# Autodesk Inventor assembly: FrontWheelForkAssembly
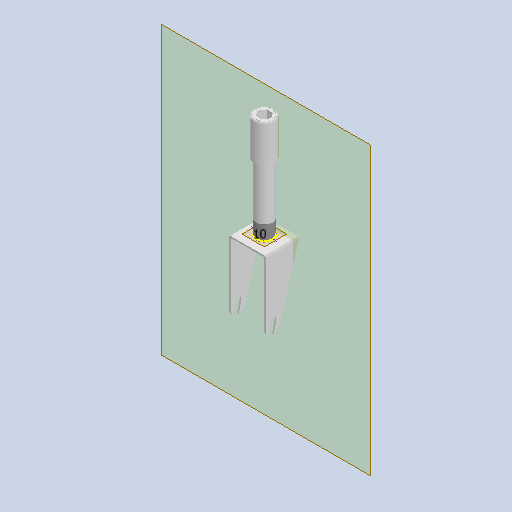
[picture p0: Inventor's stored thumbnail of the model, 512x512]
Saved by Autodesk Inventor 2022.2 (Build 262287000, 287)
## iProperties
Created: 2022-04-13
Part Number: FrontWheelForkAssembly
Document SubType Name: Assembly
Designer: foriw
Mass: 127.99 g
Surface Area: 764.001 cm^2
Volume: 122.116 cm^3
Density: 1.0481 g/cm^3
Author: foriw
## Documents named in this file (6)
- H:\inventor ting\Mekatronik beercart git\Beercart CAD\Workspaces\Workspace\FrontWheelForkAssembly.iam
- H:\inventor ting\Mekatronik beercart git\Beercart CAD\Workspaces\Workspace\Solid2.ipt
- H:\inventor ting\Mekatronik beercart git\Beercart CAD\Workspaces\Workspace\Solid3.ipt
- H:\inventor ting\Mekatronik beercart git\Beercart CAD\Libraries\Content Center Files\en-US\ISO 4762(2)\ISO 4762 - M5 x 12ISO.ipt
- H:\inventor ting\Mekatronik beercart git\Beercart CAD\Libraries\Content Center Files\en-US\ISO 4762(2)\ISO 4762 - M5 x 8ISO.ipt
- H:\inventor ting\Mekatronik beercart git\Beercart CAD\Workspaces\Workspace\Fork lower hole plate.ipt
## Components (5 placed, 5 different names)
1. ForkUpperTube — Mate:1, Mate:3, Mate:5, Mate:6
2. ForkLowerTireMount — Mate:2, Mate:4, Mate:5, Mate:6
3. ISO 4762 M5 x 12:1 — Mate:1, Mate:2
4. ISO 4762 M5 x 8:1 — Mate:3, Mate:4
5. Fork lower hole plate:1
## Relationships (6: Mate 6)
- Mate:1: ForkUpperTube ↔ ISO 4762 M5 x 12:1
- Mate:2: ForkLowerTireMount ↔ ISO 4762 M5 x 12:1
- Mate:3: ForkUpperTube ↔ ISO 4762 M5 x 8:1
- Mate:4: ForkLowerTireMount ↔ ISO 4762 M5 x 8:1
- Mate:5: ForkUpperTube ↔ ForkLowerTireMount
- Mate:6: ForkUpperTube ↔ ForkLowerTireMount
